# Autodesk Inventor assembly: Turret Shooter Assembly
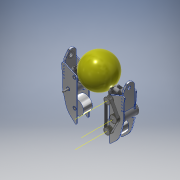
[picture p0: Inventor's stored thumbnail of the model, 180x180]
Saved by Autodesk Inventor 2019.4 (Build 234330000, 330)
## iProperties
Created: 2020-01-06
Part Number: Turret Shooter Assembly
Document SubType Name: Assembly
Designer: admin
Mass: 4067.01 g
Surface Area: 6466.54 cm^2
Volume: 4994.12 cm^3
Density: 0.814359 g/cm^3
Author: admin
## Documents named in this file (13)
- C:\Users\admin\Desktop\FRC 2020 Engineering\GitHub\7738-2020\Turret\Turret Shooter Assembly.iam
- C:\Users\admin\Desktop\FRC 2020 Engineering\GitHub\7738-2020\Turret\Omni Wheel\3_25_Omni-Directional_Wheel_217-4775.iam
- C:\Users\admin\Desktop\FRC 2020 Engineering\GitHub\7738-2020\Power Cell.ipt
- C:\Users\admin\Desktop\FRC 2020 Engineering\GitHub\7738-2020\Turret\Flywheel.ipt
- C:\Users\admin\Desktop\FRC 2020 Engineering\GitHub\7738-2020\Turret\Mini CIM\Mini_CIM_Motor_217-3371.ipt
- C:\Users\admin\Desktop\FRC 2020 Engineering\GitHub\7738-2020\CAD\Gearbox\F6800.ipt
- C:\Users\admin\Desktop\FRC 2020 Engineering\GitHub\7738-2020\Turret\Flywheel Bracket 1.ipt
- C:\Users\admin\Desktop\FRC 2020 Engineering\GitHub\7738-2020\Turret\Flywheel Bracket 2.ipt
- C:\Users\admin\Desktop\FRC 2020 Engineering\GitHub\7738-2020\Turret\Pivot Plate.ipt
- C:\Users\admin\Desktop\FRC 2020 Engineering\GitHub\7738-2020\Turret\Turret Shooter Assembly\Design Accelerator\Synchronous Belts Transmission1.iam
- C:\Users\admin\Desktop\FRC 2020 Engineering\GitHub\7738-2020\Turret\Slewing Bearing.ipt
- C:\Users\admin\Desktop\FRC 2020 Engineering\GitHub\7738-2020\CAD\Gearbox\F6804.ipt
- C:\Users\admin\Desktop\FRC 2020 Engineering\GitHub\7738-2020\Turret\Pivot Plate Idle.ipt
## Components (24 placed, 12 different names)
1. 3_25_Omni-Directional_Wheel_217-4775:1 [sub-assembly] — Angle:1, Mate:17, Flush:7, Flush:8
2. Power Cell:1 — Mate:5, Mate:6
3. Flywheel:1 — Flush:3, Mate:3, Flush:6, Mate:8, Flush:7, Mate:20, Mate:24
4. Mini_CIM_Motor_217-3371:1 — Flush:3, Mate:9, Mate:10, Mate:21, Mate:64
5. F6800:2 — Mate:11, Mate:12
6. Flywheel Bracket 1:1 — Mate:8, Mate:9, Mate:10, Mate:11, Mate:12, Mate:25, Mate:27, Mate:29, Mate:30, Mate:31
7. Flywheel Bracket 2:1 — Mate:20, Mate:21, Mate:22, Mate:23, Mate:26, Mate:28, Angle:2, Flush:9
8. F6800:3 — Mate:22, Mate:23, Mate:24
9. F6800:4 — Mate:26, Mate:28, Mate:32
10. F6800:5 — Mate:25, Mate:27
11. Pivot Plate:1 — Mate:29, Mate:30, Mate:31, Flush:10
12. Synchronous Belts Transmission:1 [sub-assembly]
13. Slewing Bearing:1
14. F6804:2 — Mate:65, Mate:66
15. 3_25_Omni-Directional_Wheel_217-4775:2 [sub-assembly] — Mate:57, Flush:8, Mate:59
16. Flywheel:2 — Mate:45, Mate:46, Mate:60, Mate:62
17. F6800:6 — Mate:46, Mate:53, Mate:55, Mate:62
18. F6800:7 — Mate:48, Mate:50, Mate:51
19. F6800:8 — Mate:54, Mate:56, Mate:57, Mate:59
20. F6800:9 — Mate:45, Mate:47, Mate:49, Mate:60
21. Mini_CIM_Motor_217-3371:2 — Mate:52, Mate:61, Mate:63, Mate:64
22. Flywheel Bracket 2:2 — Mate:47, Mate:48, Mate:49, Mate:50, Mate:51, Mate:52, Flush:9, Angle:3, Mate:68, Mate:69
23. Flywheel Bracket 1:2 — Mate:53, Mate:54, Mate:55, Mate:56, Mate:61, Mate:63, Mate:67
24. Pivot Plate Idle:1 — Mate:65, Mate:66, Mate:67, Mate:68, Mate:69, Flush:10
## Relationships (56: Mate 46, Flush 7, Angle 3)
- Flush:3 (-5 mm): Flywheel:1 ↔ Mini_CIM_Motor_217-3371:1
- Mate:3 (103.5 mm): Flywheel:1
- Mate:5: Power Cell:1
- Mate:6: Power Cell:1
- Flush:5 (103.5 mm)
- Flush:6 (-25 mm): Flywheel:1
- Mate:8: Flywheel:1 ↔ Flywheel Bracket 1:1
- Mate:9: Mini_CIM_Motor_217-3371:1 ↔ Flywheel Bracket 1:1
- Mate:10: Mini_CIM_Motor_217-3371:1 ↔ Flywheel Bracket 1:1
- Mate:11: F6800:2 ↔ Flywheel Bracket 1:1
- Mate:12 (0.2 mm): F6800:2 ↔ Flywheel Bracket 1:1
- Angle:1 (0 deg): 3_25_Omni-Directional_Wheel_217-4775:1
- Mate:17: 3_25_Omni-Directional_Wheel_217-4775:1
- Flush:7 (5.95 mm): 3_25_Omni-Directional_Wheel_217-4775:1 ↔ Flywheel:1
- Mate:20: Flywheel:1 ↔ Flywheel Bracket 2:1
- Mate:21: Mini_CIM_Motor_217-3371:1 ↔ Flywheel Bracket 2:1
- Mate:22: Flywheel Bracket 2:1 ↔ F6800:3
- Mate:23 (0.2 mm): Flywheel Bracket 2:1 ↔ F6800:3
- Mate:24 (5 mm): Flywheel:1 ↔ F6800:3
- Mate:25: Flywheel Bracket 1:1 ↔ F6800:5
- Mate:26: Flywheel Bracket 2:1 ↔ F6800:4
- Mate:27 (0.2 mm): Flywheel Bracket 1:1 ↔ F6800:5
- Mate:28 (0.2 mm): Flywheel Bracket 2:1 ↔ F6800:4
- Mate:29 (0.1 mm): Flywheel Bracket 1:1 ↔ Pivot Plate:1
- Mate:30: Flywheel Bracket 1:1 ↔ Pivot Plate:1
- Mate:31: Flywheel Bracket 1:1 ↔ Pivot Plate:1
- Mate:32: F6800:4
- Angle:2 (180 deg): Flywheel Bracket 2:1
- Mate:45 (5 mm): Flywheel:2 ↔ F6800:9
- Mate:46 (5 mm): Flywheel:2 ↔ F6800:6
- Mate:47: F6800:9 ↔ Flywheel Bracket 2:2
- Mate:48: F6800:7 ↔ Flywheel Bracket 2:2
- Mate:49 (0.2 mm): F6800:9 ↔ Flywheel Bracket 2:2
- Mate:50: F6800:7 ↔ Flywheel Bracket 2:2
- Mate:51 (0.2 mm): F6800:7 ↔ Flywheel Bracket 2:2
- Mate:52: Mini_CIM_Motor_217-3371:2 ↔ Flywheel Bracket 2:2
- Mate:53: F6800:6 ↔ Flywheel Bracket 1:2
- Mate:54: F6800:8 ↔ Flywheel Bracket 1:2
- Mate:55 (0.2 mm): F6800:6 ↔ Flywheel Bracket 1:2
- Mate:56 (0.2 mm): F6800:8 ↔ Flywheel Bracket 1:2
- Mate:57: 3_25_Omni-Directional_Wheel_217-4775:2 ↔ F6800:8
- Flush:8: 3_25_Omni-Directional_Wheel_217-4775:1 ↔ 3_25_Omni-Directional_Wheel_217-4775:2
- Flush:9: Flywheel Bracket 2:1 ↔ Flywheel Bracket 2:2
- Mate:59: 3_25_Omni-Directional_Wheel_217-4775:2 ↔ F6800:8
- Mate:60: Flywheel:2 ↔ F6800:9
- Mate:61: Mini_CIM_Motor_217-3371:2 ↔ Flywheel Bracket 1:2
- Mate:62: Flywheel:2 ↔ F6800:6
- Mate:63: Mini_CIM_Motor_217-3371:2 ↔ Flywheel Bracket 1:2
- Mate:64 (278.846 mm): Mini_CIM_Motor_217-3371:1 ↔ Mini_CIM_Motor_217-3371:2
- Angle:3 (0 deg): Flywheel Bracket 2:2
- Mate:65: F6804:2 ↔ Pivot Plate Idle:1
- Mate:66 (0.2 mm): F6804:2 ↔ Pivot Plate Idle:1
- Mate:67 (0.2 mm): Flywheel Bracket 1:2 ↔ Pivot Plate Idle:1
- Mate:68: Flywheel Bracket 2:2 ↔ Pivot Plate Idle:1
- Mate:69: Flywheel Bracket 2:2 ↔ Pivot Plate Idle:1
- Flush:10: Pivot Plate:1 ↔ Pivot Plate Idle:1
